# Autodesk Inventor assembly: Ramie_z
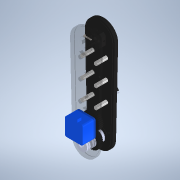
[picture p0: Inventor's stored thumbnail of the model, 180x180]
Saved by Autodesk Inventor 2021 (Build 250183000, 183)
## iProperties
Created: 2021-07-30
Part Number: Ramie_z
Document SubType Name: Assembly
Designer: Janusz
Author: Janusz
Revision Number: ANY
## Documents named in this file (12)
- D:\ROBOT\Ramie_z.iam
- D:\ROBOT\Ramie_Na silnik.ipt
- D:\ROBOT\Ramie.ipt
- D:\ROBOT\silnik2_kserokopiarka_bez_blaszki.ipt
- D:\ROBOT\Obudowa_ramienia.ipt
- D:\ROBOT\rod_8mm_29 mm.ipt
- D:\ROBOT\Zêbatka_silnik_ksero_ISO - RH Helical gear 0.9M 30T 45HA 20PA 10FW ---30A75H50L12.0N.ipt
- D:\ROBOT\³o¿ysko_oporowe_12x26x9.ipt
- D:\ROBOT\Zêbatka_ramie_walek_ISO - RH Helical gear 0.9M 30T 45HA 20PA 8FW ---30C20H20L8.0N.ipt
- D:\ROBOT\ISO 10642 - M3 x 10 - 10N_ISO 10642 - M3 x 10 - 10N.ipt
- D:\ROBOT\ISO 10642 - M3 x 16 - 16N_ISO 10642 - M3 x 16 - 16N.ipt
- D:\ROBOT\MicroSwitchButton2.ipt
## Components (20 placed, 20 different names)
1. Ramie_Na silnik_56 — Zestawiające:1, Zestawiające:2, Zestawiające:13, Zestawiające:14, Zestawiające:15, Zestawiające:20, Zestawiające:21, Równoległe:1, Zestawiające:23, Zestawiające:24, Zestawiające:25, Zestawiające:33
2. Ramie_57 — Zestawiające:9, Zestawiające:10, Zestawiające:16, Zestawiające:17, Zestawiające:23, Zestawiające:24, Zestawiające:25, Zestawiające:26, Zestawiające:27, Zestawiające:28, Zestawiające:29, Zestawiające:30, Zestawiające:31, Zestawiające:32, Zestawiające:34, Zestawiające:35, Zestawiające:36, Zestawiające:37, Zestawiające:38, Zestawiające:39
3. silnik2_kserokopiarka_bez_blaszki_58 — Zestawiające:13, Zestawiające:14, Zestawiające:15, Równoległe:41, Zestawiające:40
4. Obudowa_ramienia_59
5. rod_8mm_29 mm_60 — Równoległe:5, Równoległe:6, Zestawiające:29
6. rod_8mm_29 mm_61 — Równoległe:2, Równoległe:3, Zestawiające:28
7. rod_8mm_29 mm_62 — Równoległe:2, Równoległe:4, Zestawiające:26, Zestawiające:32
8. rod_8mm_29 mm_63 — Równoległe:4, Równoległe:5, Zestawiające:27
9. rod_8mm_29 mm_64 — Równoległe:6, Zestawiające:31
10. rod_8mm_29 mm_65 — Równoległe:3, Zestawiające:30
11. Zêbatka_silnik_ksero_ISO - RH Helical gear 0.9M 30T 45HA 20PA 10FW ---30A75H50L12.0N_66 — Równoległe:41, Zestawiające:40
12. ³o¿ysko_oporowe_12x26x9_67 — Zestawiające:1, Zestawiające:2
13. Zêbatka_ramie_walek_ISO - RH Helical gear 0.9M 30T 45HA 20PA 8FW ---30C20H20L8.0N_68 — Zestawiające:5, Zestawiające:6, Zestawiające:7, Zestawiające:8, Zestawiające:22, Styczny:1
14. ³o¿ysko_oporowe_12x26x9_69 — Zestawiające:16, Zestawiające:17
15. ³o¿ysko_oporowe_12x26x9_70 — Zestawiające:6, Zestawiające:8, Zestawiające:9, Zestawiające:10
16. ³o¿ysko_oporowe_12x26x9_71 — Zestawiające:5, Zestawiające:7
17. ISO 10642 - M3 x 10 - 10N_ISO 10642 - M3 x 10 - 10N_74 — Zestawiające:22, Styczny:1
18. ISO 10642 - M3 x 16 - 16N_ISO 10642 - M3 x 16 - 16N_75 — Zestawiające:33
19. MicroSwitchButton2_76 — Zestawiające:37, Zestawiające:38, Zestawiające:39
20. MicroSwitchButton2_77 — Zestawiające:34, Zestawiające:35, Zestawiające:36
## Relationships (42: Mate 34, Flush 7, Tangent 1)
- Zestawiające:1 [Mate]: Ramie_Na silnik_56 ↔ ³o¿ysko_oporowe_12x26x9_67
- Zestawiające:2 [Mate]: Ramie_Na silnik_56 ↔ ³o¿ysko_oporowe_12x26x9_67
- Zestawiające:5 [Mate]: Zêbatka_ramie_walek_ISO - RH Helical gear 0.9M 30T 45HA 20PA 8FW ---30C20H20L8.0N_68 ↔ ³o¿ysko_oporowe_12x26x9_71
- Zestawiające:6 [Mate]: Zêbatka_ramie_walek_ISO - RH Helical gear 0.9M 30T 45HA 20PA 8FW ---30C20H20L8.0N_68 ↔ ³o¿ysko_oporowe_12x26x9_70
- Zestawiające:7 [Mate]: Zêbatka_ramie_walek_ISO - RH Helical gear 0.9M 30T 45HA 20PA 8FW ---30C20H20L8.0N_68 ↔ ³o¿ysko_oporowe_12x26x9_71
- Zestawiające:8 [Mate]: Zêbatka_ramie_walek_ISO - RH Helical gear 0.9M 30T 45HA 20PA 8FW ---30C20H20L8.0N_68 ↔ ³o¿ysko_oporowe_12x26x9_70
- Zestawiające:9 [Mate]: Ramie_57 ↔ ³o¿ysko_oporowe_12x26x9_70
- Zestawiające:10 [Mate]: Ramie_57 ↔ ³o¿ysko_oporowe_12x26x9_70
- Zestawiające:13 [Mate]: Ramie_Na silnik_56 ↔ silnik2_kserokopiarka_bez_blaszki_58
- Zestawiające:14 [Mate]: Ramie_Na silnik_56 ↔ silnik2_kserokopiarka_bez_blaszki_58
- Zestawiające:15 [Mate]: Ramie_Na silnik_56 ↔ silnik2_kserokopiarka_bez_blaszki_58
- Zestawiające:16 [Mate]: Ramie_57 ↔ ³o¿ysko_oporowe_12x26x9_69
- Zestawiające:17 [Mate]: Ramie_57 ↔ ³o¿ysko_oporowe_12x26x9_69
- Zestawiające:20 [Mate]: Ramie_Na silnik_56
- Zestawiające:21 [Mate]: Ramie_Na silnik_56
- Równoległe:1 [Flush]: Ramie_Na silnik_56
- Zestawiające:22 [Mate]: Zêbatka_ramie_walek_ISO - RH Helical gear 0.9M 30T 45HA 20PA 8FW ---30C20H20L8.0N_68 ↔ ISO 10642 - M3 x 10 - 10N_ISO 10642 - M3 x 10 - 10N_74
- Styczny:1 [Tangent]: Zêbatka_ramie_walek_ISO - RH Helical gear 0.9M 30T 45HA 20PA 8FW ---30C20H20L8.0N_68 ↔ ISO 10642 - M3 x 10 - 10N_ISO 10642 - M3 x 10 - 10N_74
- Zestawiające:23 [Mate]: Ramie_Na silnik_56 ↔ Ramie_57
- Zestawiające:24 [Mate]: Ramie_Na silnik_56 ↔ Ramie_57
- Zestawiające:25 [Mate]: Ramie_Na silnik_56 ↔ Ramie_57
- Równoległe:2 [Flush]: rod_8mm_29 mm_61 ↔ rod_8mm_29 mm_62
- Równoległe:3 [Flush]: rod_8mm_29 mm_61 ↔ rod_8mm_29 mm_65
- Równoległe:4 [Flush]: rod_8mm_29 mm_62 ↔ rod_8mm_29 mm_63
- Równoległe:5 [Flush]: rod_8mm_29 mm_60 ↔ rod_8mm_29 mm_63
- Równoległe:6 [Flush]: rod_8mm_29 mm_60 ↔ rod_8mm_29 mm_64
- Zestawiające:26 [Mate]: Ramie_57 ↔ rod_8mm_29 mm_62
- Zestawiające:27 [Mate]: Ramie_57 ↔ rod_8mm_29 mm_63
- Zestawiające:28 [Mate]: Ramie_57 ↔ rod_8mm_29 mm_61
- Zestawiające:29 [Mate]: Ramie_57 ↔ rod_8mm_29 mm_60
- Zestawiające:30 [Mate]: Ramie_57 ↔ rod_8mm_29 mm_65
- Zestawiające:31 [Mate]: Ramie_57 ↔ rod_8mm_29 mm_64
- Zestawiające:32 [Mate] (2 mm): Ramie_57 ↔ rod_8mm_29 mm_62
- Zestawiające:33 [Mate]: Ramie_Na silnik_56 ↔ ISO 10642 - M3 x 16 - 16N_ISO 10642 - M3 x 16 - 16N_75
- Zestawiające:34 [Mate]: Ramie_57 ↔ MicroSwitchButton2_77
- Zestawiające:35 [Mate]: Ramie_57 ↔ MicroSwitchButton2_77
- Zestawiające:36 [Mate]: Ramie_57 ↔ MicroSwitchButton2_77
- Zestawiające:37 [Mate]: Ramie_57 ↔ MicroSwitchButton2_76
- Zestawiające:38 [Mate]: Ramie_57 ↔ MicroSwitchButton2_76
- Zestawiające:39 [Mate]: Ramie_57 ↔ MicroSwitchButton2_76
- Równoległe:41 [Flush]: silnik2_kserokopiarka_bez_blaszki_58 ↔ Zêbatka_silnik_ksero_ISO - RH Helical gear 0.9M 30T 45HA 20PA 10FW ---30A75H50L12.0N_66
- Zestawiające:40 [Mate]: silnik2_kserokopiarka_bez_blaszki_58 ↔ Zêbatka_silnik_ksero_ISO - RH Helical gear 0.9M 30T 45HA 20PA 10FW ---30A75H50L12.0N_66
